# Autodesk Inventor assembly: measuring_test
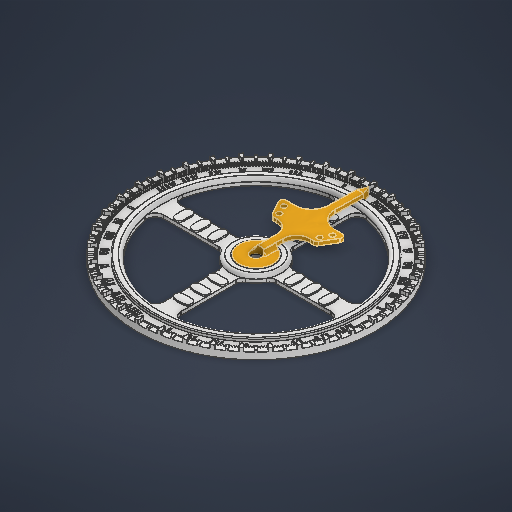
[picture p0: Inventor's stored thumbnail of the model, 512x512]
Saved by Autodesk Inventor 2026.1 (Build 301233000, 233)
## iProperties
Created: 2025-12-25
Part Number: measuring_test
Document SubType Name: Assembly
Designer: emanuel
Author: emanuel
## Documents named in this file (3)
- C:\Users\emanuel\UnFolder\SpiderRobo\3dmodel\measuring_test.iam
- C:\Users\emanuel\UnFolder\SpiderRobo\3dmodel\measuring_disk.ipt
- C:\Users\emanuel\UnFolder\SpiderRobo\3dmodel\measuring_triangle.ipt
## Components (2 placed, 2 different names)
1. measuring_disk:1 — Mate:13, Mate:14
2. measuring_triangle:1 — Mate:13, Mate:14
## Relationships (2: Mate 2)
- Mate:13: measuring_disk:1 ↔ measuring_triangle:1
- Mate:14: measuring_disk:1 ↔ measuring_triangle:1
